# Autodesk Inventor assembly: 000.100 - Electronic box
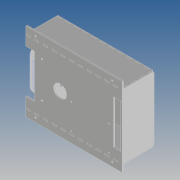
[picture p0: Inventor's stored thumbnail of the model, 180x180]
Saved by Autodesk Inventor 2020 (Build 240168000, 168)
## iProperties
Created: 2021-06-27
Part Number: 000.100 - Electronic box
Document SubType Name: Assembly
Designer: Петров Иван
Mass: 980.412 g
Surface Area: 4009.02 cm^2
Volume: 569.609 cm^3
Density: 1.7212 g/cm^3
Author: Петров Иван
## Documents named in this file (10)
- E:\IVAN\Ivan_desktop\My_projects\Test Robots\4wheel\viki_mchs_robot\000.100 - Electronic box.iam
- E:\IVAN\Ivan_desktop\My_projects\Test Robots\4wheel\viki_mchs_robot\000.101 - Bottom.ipt
- E:\IVAN\Ivan_desktop\My_projects\Test Robots\4wheel\viki_mchs_robot\standart_components\JetsonNano\Jetson nano_fixed.iam
- E:\IVAN\Ivan_desktop\My_projects\Test Robots\4wheel\viki_mchs_robot\standart_components\Raspberry Pi 4B\Raspberry-Pi-4-Model-B-03.ipt
- E:\IVAN\Ivan_desktop\My_projects\Test Robots\4wheel\viki_mchs_robot\standart_components\tests\realsenses_plate_v2.ipt.iam
- E:\IVAN\Ivan_desktop\My_projects\Test Robots\4wheel\viki_mchs_robot\000.102 - Left wall.ipt
- E:\IVAN\Ivan_desktop\My_projects\Test Robots\4wheel\viki_mchs_robot\000.103 - Right wall.ipt
- E:\IVAN\Ivan_desktop\My_projects\Test Robots\4wheel\viki_mchs_robot\000.104 - Back wall.ipt
- E:\IVAN\Ivan_desktop\My_projects\Test Robots\4wheel\viki_mchs_robot\000.104 - Cap.ipt
- realsenses_plate_v2.ipt
## Components (8 placed, 8 different names)
1. 000.101 - Bottom:1 — Заподлицо:1, Совмещение:1, Заподлицо:2, Заподлицо:4, Совмещение:2, Заподлицо:5, Заподлицо:6, Совмещение:3, Заподлицо:7, Совмещение:4, Заподлицо:8, Заподлицо:9, Заподлицо:10
2. Jetson nano_fixed:1 [sub-assembly] — Заподлицо:2, Заподлицо:4, Совмещение:2
3. Raspberry-Pi-4-Model-B-03:1
4. realsenses_plate_v2.ipt:1 [sub-assembly] — Заподлицо:1, Совмещение:1, Заподлицо:5
5. 000.102 - Left wall:1 — Заподлицо:6, Совмещение:3, Заподлицо:7
6. 000.103 - Right wall:1 — Совмещение:4, Заподлицо:8, Заподлицо:9, Совмещение:5, Заподлицо:11, Заподлицо:12, Заподлицо:13, Заподлицо:14
7. 000.104 - Back wall:1 — Совмещение:5, Заподлицо:10, Заподлицо:11
8. 000.104 - Cap:1 — Заподлицо:12, Заподлицо:13, Заподлицо:14
## Relationships (18: Flush 13, Mate 5)
- Заподлицо:1 [Flush] (4 mm): 000.101 - Bottom:1 ↔ realsenses_plate_v2.ipt:1
- Совмещение:1 [Mate]: 000.101 - Bottom:1 ↔ realsenses_plate_v2.ipt:1
- Заподлицо:2 [Flush] (20 mm): 000.101 - Bottom:1 ↔ Jetson nano_fixed:1
- Заподлицо:4 [Flush] (20 mm): 000.101 - Bottom:1 ↔ Jetson nano_fixed:1
- Совмещение:2 [Mate] (5 mm): 000.101 - Bottom:1 ↔ Jetson nano_fixed:1
- Заподлицо:5 [Flush] (32.5 mm): 000.101 - Bottom:1 ↔ realsenses_plate_v2.ipt:1
- Заподлицо:6 [Flush]: 000.101 - Bottom:1 ↔ 000.102 - Left wall:1
- Совмещение:3 [Mate]: 000.101 - Bottom:1 ↔ 000.102 - Left wall:1
- Заподлицо:7 [Flush]: 000.101 - Bottom:1 ↔ 000.102 - Left wall:1
- Совмещение:4 [Mate]: 000.101 - Bottom:1 ↔ 000.103 - Right wall:1
- Заподлицо:8 [Flush]: 000.101 - Bottom:1 ↔ 000.103 - Right wall:1
- Заподлицо:9 [Flush]: 000.101 - Bottom:1 ↔ 000.103 - Right wall:1
- Совмещение:5 [Mate]: 000.103 - Right wall:1 ↔ 000.104 - Back wall:1
- Заподлицо:10 [Flush]: 000.101 - Bottom:1 ↔ 000.104 - Back wall:1
- Заподлицо:11 [Flush]: 000.103 - Right wall:1 ↔ 000.104 - Back wall:1
- Заподлицо:12 [Flush]: 000.103 - Right wall:1 ↔ 000.104 - Cap:1
- Заподлицо:13 [Flush]: 000.103 - Right wall:1 ↔ 000.104 - Cap:1
- Заподлицо:14 [Flush]: 000.103 - Right wall:1 ↔ 000.104 - Cap:1
